# Autodesk Inventor assembly: hotend
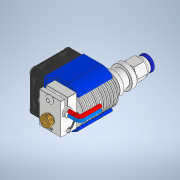
[picture p0: Inventor's stored thumbnail of the model, 180x180]
Saved by Autodesk Inventor 2020.3 (Build 243373000, 373)
## iProperties
Created: 2021-08-09
Part Number: hotend
Document SubType Name: Assembly
Designer: szymo
Author: szymo
## Documents named in this file (3)
- E:\Dropbox_backup\solidworks\ender5plus\czesci_dodane\direct\hotend_v6\hotend.iam
- E:\Dropbox_backup\solidworks\ender5plus\czesci_dodane\direct\hotend_v6\heat_block.ipt
- E:\Dropbox_backup\solidworks\ender5plus\czesci_dodane\direct\hotend_v6\radiator.ipt
## Components (2 placed, 2 different names)
1. heat_block:1 — Zestawiające:1, Zestawiające:2, Zestawiające:3, Kątowe:1
2. radiator:1 — Zestawiające:1, Zestawiające:2, Zestawiające:3, Kątowe:1
## Relationships (4: Mate 3, Angle 1)
- Zestawiające:1 [Mate]: heat_block:1 ↔ radiator:1
- Zestawiające:2 [Mate] (2 mm): heat_block:1 ↔ radiator:1
- Zestawiające:3 [Mate]: heat_block:1 ↔ radiator:1
- Kątowe:1 [Angle] (0 deg): heat_block:1 ↔ radiator:1
